# Autodesk Inventor assembly: base_link
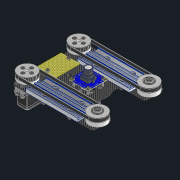
[picture p0: Inventor's stored thumbnail of the model, 180x180]
Saved by Autodesk Inventor 2021 (Build 250183000, 183)
## iProperties
Created: 2021-08-10
Part Number: base_link
Document SubType Name: Assembly
Designer: yuta0
Author: yuta0
## Documents named in this file (2)
- C:\Users\yuta0\Documents\GitHub\catchrobo_hardware\mesh\base_link.iam
- C:\Users\yuta0\Documents\GitHub\catchrobo_hardware\assy-robot\s-assy-gripper_without_finger.iam
## Components (1 placed, 1 different names)
1. s-assy-gripper_without_finger:1 [sub-assembly] — メイト:1
## Relationships (1: Mate 1)
- メイト:1 [Mate]: s-assy-gripper_without_finger:1
